# Autodesk Inventor assembly: 300069
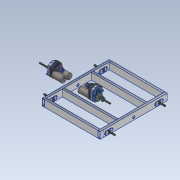
[picture p0: Inventor's stored thumbnail of the model, 180x180]
Saved by Autodesk Inventor 2020 (Build 240168000, 168)
## iProperties
Created: 2021-11-02
Part Number: 300069
Document SubType Name: Assembly
Designer: Byron Robotics
Mass: 9925.38 g
Surface Area: 24660.2 cm^2
Volume: 5223.25 cm^3
Density: 1.90023 g/cm^3
Author: Byron Robotics
Revision Number: A
## Documents named in this file (6)
- C:\$WorkingFolder\Projects\2022\Drivebase\300069.iam
- C:\$WorkingFolder\Projects\2022\Drivebase\300064.iam
- C:\$WorkingFolder\Projects\2022\Drivebase\3 Stage Ball Shifter Assembly\3 Stage with Grayhill Encoder (217-2615).iam
- C:\$WorkingFolder\Projects\2021\2020 robot base\2020 p-am-3999 17T 25 Chain Double Sprocket For WCD.ipt
- C:\$WorkingFolder\Projects\2022\Drivebase\300072.iam
- C:\$WorkingFolder\Projects\2022\Drivebase\Drivebase Parametric Spreadsheet.xlsx
## Components (9 placed, 4 different names)
1. 300064:1 [sub-assembly] — Mate:2, Mate:3, Mate:4, Mate:5, Slider:1, Slider:2, Slider:3, Slider:4
2. 3 Stage with Grayhill Encoder (217-2615):1 [sub-assembly] — Mate:2
3. 3 Stage with Grayhill Encoder (217-2615):2 [sub-assembly] — Mate:5
4. 2020 p-am-3999 17T 25 Chain Double Sprocket For WCD:1 — Mate:3
5. 2020 p-am-3999 17T 25 Chain Double Sprocket For WCD:2 — Mate:4
6. 300072:1 [sub-assembly] — Slider:3
7. 300072:2 [sub-assembly] — Slider:2
8. 300072:3 [sub-assembly] — Slider:4
9. 300072:4 [sub-assembly] — Slider:1
## Relationships (8: Mate 4, TranslationJoint 4)
- Mate:2: 300064:1 ↔ 3 Stage with Grayhill Encoder (217-2615):1
- Mate:3: 300064:1 ↔ 2020 p-am-3999 17T 25 Chain Double Sprocket For WCD:1
- Mate:4: 300064:1 ↔ 2020 p-am-3999 17T 25 Chain Double Sprocket For WCD:2
- Mate:5: 300064:1 ↔ 3 Stage with Grayhill Encoder (217-2615):2
- Slider:1 [TranslationJoint]: 300064:1 ↔ 300072:4
- Slider:2 [TranslationJoint]: 300064:1 ↔ 300072:2
- Slider:3 [TranslationJoint]: 300064:1 ↔ 300072:1
- Slider:4 [TranslationJoint]: 300064:1 ↔ 300072:3
## Named parameters: DrivebaseLength = 762 mm, DrivebaseWidth = 660.4 mm, CenterlineDrivebaseLength = 736.6 mm, CenterlineDrivebaseWidth = 635 mm, ShapeHeight = 76.2 mm, ShapeWidth = 25.4 mm, ShapeThickness = 3.175 mm, WheelDiameter = 152.4 mm, WheelRadius = 76.2 mm, WheelClearancetoFrame = 25.4 mm, WheelDistanceFromEdge = 101.6 mm, SlotLength = 88.9 mm, SlotWidth = 15.9512 mm, CenterAxleDrop = 3.175 mm, CenterAxleXPosition = 381 mm, CenterAxleYPosition = 25.4 mm, Crossmember1Position = 203.2 mm, Crossmember2Position = 203.2 mm, TensionAssemblyJointTravelLengthStart = -15.875 mm, SlidingTensionerRoundClearance = 0.0762 mm, CenterPointToTensionerRound = 28.575 mm, SlidingTensionerRoundDiameter = 15.875 mm, TensionAssemblyJointTravelLengthEnd = 15.875 mm
